# Autodesk Inventor assembly: stage1Mount
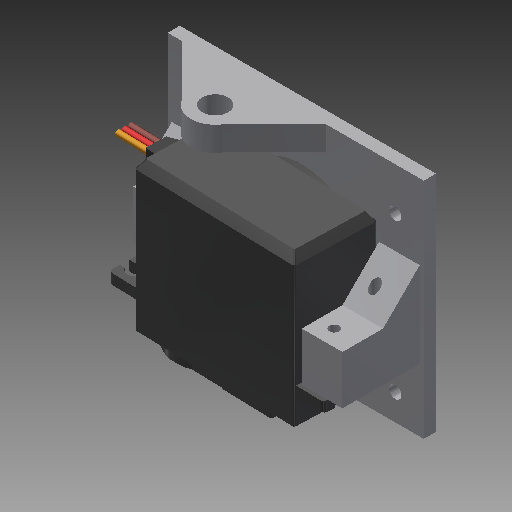
[picture p0: Inventor's stored thumbnail of the model, 512x512]
Saved by Autodesk Inventor 2017 (Build 210142000, 142)
## iProperties
Created: 2017-03-10
Part Number: stage1Mount
Description: FreeCAD Model
Document SubType Name: Assembly
Designer: Naga
Authority: Unknown
Title: E:/GDrive/IEEE CS/SoutheastCon2017/Cad/tilt/step/tiltservomount_std.step
Author: Author
## Documents named in this file (3)
- E:\GDrive\IEEE CS\SoutheastCon2017\Cad\tilt\step\stage1Mount.iam
- E:\GDrive\IEEE CS\SoutheastCon2017\Cad\Motors\MG995_Servo.iam
- E:\GDrive\IEEE CS\SoutheastCon2017\Cad\tilt\step\tiltProbe.ipt
## Components (2 placed, 2 different names)
1. 3 — Mate:1, Mate:2, Mate:3
2. MG995_Servo:1 [sub-assembly] — Mate:1, Mate:2, Mate:3
## Relationships (3: Mate 3)
- Mate:1: 3 ↔ MG995_Servo:1
- Mate:2: 3 ↔ MG995_Servo:1
- Mate:3: 3 ↔ MG995_Servo:1
